# Autodesk Inventor assembly: licht_200
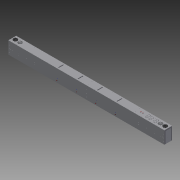
[picture p0: Inventor's stored thumbnail of the model, 180x180]
Saved by Autodesk Inventor 2015 (Build 190159000, 159)
## iProperties
Created: 2018-02-17
Part Number: licht_200
Document SubType Name: Assembly
Designer: wepet
Author: wepet
## Documents named in this file (13)
- C:\workspace\robosax\licht\Einzelteil_200\licht_200.iam
- C:\workspace\robosax\licht\Einzelteil_200\licht_200_back.ipt
- C:\workspace\robosax\licht\Einzelteil_200\licht_200_front.ipt
- C:\workspace\robosax\licht\Einzelteil_200\licht_200_top_teil_a.ipt
- C:\workspace\robosax\licht\Einzelteil_200\licht_200_top_teil_b.ipt
- C:\workspace\robosax\licht\Einzelteil_200\licht_200_side_middle.ipt
- C:\workspace\robosax\licht\Einzelteil_200\licht_200_support.ipt
- C:\workspace\robosax\licht\Einzelteil_200\licht_200_side_left.ipt
- C:\workspace\robosax\licht\Einzelteil_200\licht_200_side_right.ipt
- C:\workspace\robosax\licht\Zusatzelemente\licht_led_blau.ipt
- C:\workspace\robosax\licht\Zusatzelemente\licht_taster.ipt
- C:\workspace\robosax\licht\Zusatzelemente\anschluss_strom.ipt
- C:\workspace\robosax\licht\Zusatzelemente\anschluss_daten.iam
## Components (23 placed, 12 different names)
1. licht_200_back:1 — Fluchtend:3, Fluchtend:4, Fluchtend:5, Passend:9
2. licht_200_front:1 — Passend:1, Passend:2, Passend:3, Passend:4, Fluchtend:1, Fluchtend:2, Fluchtend:3, Fluchtend:4, Passend:10, Passend:13, Passend:15, Passend:18, Passend:20, Passend:21, Fluchtend:10, Passend:23, Fluchtend:11, Einfügen:1, Einfügen:2, Einfügen:3, Einfügen:4, Einfügen:5, Einfügen:6, Einfügen:7, Einfügen:8
3. licht_200_top_teil_a:1 — Passend:4, Fluchtend:1, Fluchtend:2, Fluchtend:5, Fluchtend:6, Fluchtend:7, Passend:5, Passend:8, Passend:24, Drehbar:1, Drehbar:3, Passend:25
4. licht_200_top_teil_b:1 — Fluchtend:6, Fluchtend:7, Passend:5, Passend:22, Einfügen:9, Einfügen:10, Drehbar:2, Drehbar:4, Passend:26
5. licht_200_side_middle:1 — Passend:8, Passend:9, Passend:10
6. licht_200_support:1 — Passend:13, Passend:15
7. licht_200_support:2 — Passend:18, Passend:20
8. licht_200_side_left:1 — Passend:23, Passend:24, Fluchtend:11
9. licht_200_side_right:1 — Passend:21, Passend:22, Fluchtend:10
10. licht_led_blau:1 — Einfügen:4
11. licht_led_blau:2 — Einfügen:3
12. licht_led_blau:3 — Einfügen:1
13. licht_led_blau:4 — Einfügen:2
14. licht_taster:1 — Einfügen:5
15. licht_taster:2 — Einfügen:6
16. licht_taster:3 — Einfügen:7
17. licht_taster:4 — Einfügen:8
18. licht_taster:5 — Einfügen:9
19. licht_taster:6 — Einfügen:10
20. anschluss_strom:1 — Drehbar:1
21. anschluss_strom:2 — Drehbar:2
22. anschluss_daten:1 [sub-assembly] — Drehbar:3, Passend:25
23. anschluss_daten:2 [sub-assembly] — Drehbar:4, Passend:26
## Relationships (41: Mate 18, Insert 10, Flush 9, RevoluteJoint 4)
- Passend:1 [Mate]: licht_200_front:1
- Passend:2 [Mate]: licht_200_front:1
- Passend:3 [Mate]: licht_200_front:1
- Passend:4 [Mate]: licht_200_front:1 ↔ licht_200_top_teil_a:1
- Fluchtend:1 [Flush]: licht_200_front:1 ↔ licht_200_top_teil_a:1
- Fluchtend:2 [Flush]: licht_200_front:1 ↔ licht_200_top_teil_a:1
- Fluchtend:3 [Flush]: licht_200_back:1 ↔ licht_200_front:1
- Fluchtend:4 [Flush]: licht_200_back:1 ↔ licht_200_front:1
- Fluchtend:5 [Flush]: licht_200_back:1 ↔ licht_200_top_teil_a:1
- Fluchtend:6 [Flush]: licht_200_top_teil_a:1 ↔ licht_200_top_teil_b:1
- Fluchtend:7 [Flush]: licht_200_top_teil_a:1 ↔ licht_200_top_teil_b:1
- Passend:5 [Mate]: licht_200_top_teil_a:1 ↔ licht_200_top_teil_b:1
- Passend:8 [Mate]: licht_200_top_teil_a:1 ↔ licht_200_side_middle:1
- Passend:9 [Mate]: licht_200_back:1 ↔ licht_200_side_middle:1
- Passend:10 [Mate]: licht_200_front:1 ↔ licht_200_side_middle:1
- Passend:13 [Mate]: licht_200_front:1 ↔ licht_200_support:1
- Passend:15 [Mate]: licht_200_front:1 ↔ licht_200_support:1
- Passend:18 [Mate]: licht_200_front:1 ↔ licht_200_support:2
- Passend:20 [Mate]: licht_200_front:1 ↔ licht_200_support:2
- Passend:21 [Mate]: licht_200_front:1 ↔ licht_200_side_right:1
- Passend:22 [Mate]: licht_200_top_teil_b:1 ↔ licht_200_side_right:1
- Fluchtend:10 [Flush]: licht_200_front:1 ↔ licht_200_side_right:1
- Passend:23 [Mate]: licht_200_front:1 ↔ licht_200_side_left:1
- Passend:24 [Mate]: licht_200_top_teil_a:1 ↔ licht_200_side_left:1
- Fluchtend:11 [Flush]: licht_200_front:1 ↔ licht_200_side_left:1
- Einfügen:1 [Insert] (-5 mm): licht_200_front:1 ↔ licht_led_blau:3
- Einfügen:2 [Insert] (-5 mm): licht_200_front:1 ↔ licht_led_blau:4
- Einfügen:3 [Insert]: licht_200_front:1 ↔ licht_led_blau:2
- Einfügen:4 [Insert]: licht_200_front:1 ↔ licht_led_blau:1
- Einfügen:5 [Insert] (5 mm): licht_200_front:1 ↔ licht_taster:1
- Einfügen:6 [Insert] (5 mm): licht_200_front:1 ↔ licht_taster:2
- Einfügen:7 [Insert] (5 mm): licht_200_front:1 ↔ licht_taster:3
- Einfügen:8 [Insert] (5 mm): licht_200_front:1 ↔ licht_taster:4
- Einfügen:9 [Insert] (5 mm): licht_200_top_teil_b:1 ↔ licht_taster:5
- Einfügen:10 [Insert] (5 mm): licht_200_top_teil_b:1 ↔ licht_taster:6
- Drehbar:1 [RevoluteJoint] (-7 mm): licht_200_top_teil_a:1 ↔ anschluss_strom:1
- Drehbar:2 [RevoluteJoint] (-4.5 mm): licht_200_top_teil_b:1 ↔ anschluss_strom:2
- Drehbar:3 [RevoluteJoint]: licht_200_top_teil_a:1 ↔ anschluss_daten:1
- Passend:25 [Mate]: licht_200_top_teil_a:1 ↔ anschluss_daten:1
- Drehbar:4 [RevoluteJoint]: licht_200_top_teil_b:1 ↔ anschluss_daten:2
- Passend:26 [Mate]: licht_200_top_teil_b:1 ↔ anschluss_daten:2
